# Autodesk Inventor assembly: belt_linear
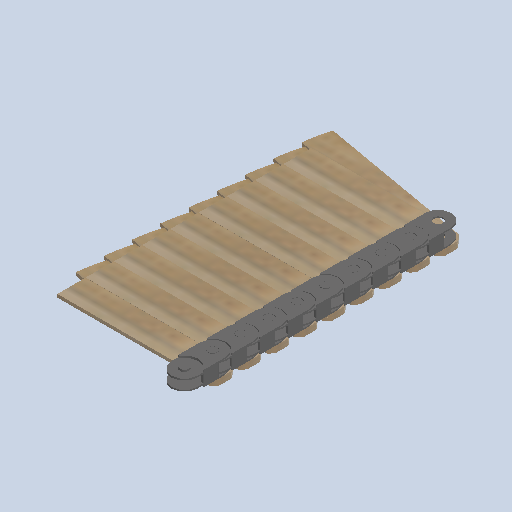
[picture p0: Inventor's stored thumbnail of the model, 512x512]
Saved by Autodesk Inventor 2024.1 (Build 281209000, 209)
## iProperties
Created: 2025-09-27
Part Number: belt_linear
Document SubType Name: Assembly
Designer: hibik
Author: hibik
## Documents named in this file (3)
- C:\Users\hibik\Documents\Robomech\conveyer\belt\belt_linear.iam
- C:\Users\hibik\Documents\Robomech\conveyer\belt\belt.ipt
- C:\Users\hibik\Documents\Robomech\conveyer\belt\dish.iam
## Components (18 placed, 2 different names)
1. belt:1 — 挿入:1, 挿入:5, 角度:1, 角度:9
2. belt:2 — 挿入:1, 挿入:2, 挿入:6, 角度:4, 角度:9, 角度:10
3. belt:3 — 挿入:2, 挿入:3, 挿入:7, 角度:3, 角度:10, 角度:11
4. belt:4 — 挿入:3, 挿入:8, 角度:2, 挿入:16, 角度:11, 角度:12
5. dish:1 [sub-assembly] — 挿入:5, 角度:1
6. dish:2 [sub-assembly] — 挿入:6, 角度:4
7. dish:3 [sub-assembly] — 挿入:7, 角度:3
8. dish:4 [sub-assembly] — 挿入:8, 角度:2
9. belt:5 — 挿入:16, 角度:12, 角度:13
10. belt:6 — 角度:13, 角度:14
11. belt:7 — 角度:14, 角度:15
12. belt:8 — 角度:15, 挿入:18, 角度:17
13. dish:5 [sub-assembly]
14. dish:6 [sub-assembly]
15. dish:7 [sub-assembly]
16. dish:8 [sub-assembly]
17. belt:9 — 挿入:18, 角度:17
18. dish:9 [sub-assembly]
## Relationships (34: Insert 17, Angle 17)
- 挿入:1 [Insert] (0.6 mm): belt:1 ↔ belt:2
- 挿入:2 [Insert] (0.6 mm): belt:2 ↔ belt:3
- 挿入:3 [Insert] (0.6 mm): belt:3 ↔ belt:4
- 挿入:5 [Insert]: belt:1 ↔ dish:1
- 角度:1 [Angle] (0 deg): belt:1 ↔ dish:1
- 挿入:6 [Insert]: belt:2 ↔ dish:2
- 挿入:7 [Insert]: belt:3 ↔ dish:3
- 挿入:8 [Insert]: belt:4 ↔ dish:4
- 角度:2 [Angle] (0 deg): belt:4 ↔ dish:4
- 角度:3 [Angle] (0 deg): belt:3 ↔ dish:3
- 角度:4 [Angle] (0 deg): belt:2 ↔ dish:2
- [Insert] (0.6 mm): belt:5 ↔ belt:6
- [Insert] (0.6 mm): belt:6 ↔ belt:7
- [Insert] (0.6 mm): belt:7 ↔ belt:8
- [Insert]: belt:5 ↔ dish:5
- [Angle] (0 deg): belt:5 ↔ dish:5
- [Insert]: belt:6 ↔ dish:6
- [Insert]: belt:7 ↔ dish:7
- [Insert]: belt:8 ↔ dish:8
- [Angle] (0 deg): belt:8 ↔ dish:8
- [Angle] (0 deg): belt:7 ↔ dish:7
- [Angle] (0 deg): belt:6 ↔ dish:6
- 挿入:16 [Insert] (0.6 mm): belt:4 ↔ belt:5
- 角度:9 [Angle] (0 deg): belt:1 ↔ belt:2
- 角度:10 [Angle] (0 deg): belt:2 ↔ belt:3
- 角度:11 [Angle] (0 deg): belt:3 ↔ belt:4
- 角度:12 [Angle] (0 deg): belt:4 ↔ belt:5
- 角度:13 [Angle] (0 deg): belt:5 ↔ belt:6
- 角度:14 [Angle] (0 deg): belt:6 ↔ belt:7
- 角度:15 [Angle] (0 deg): belt:7 ↔ belt:8
- [Insert]: belt:9 ↔ dish:9
- [Angle] (0 deg): belt:9 ↔ dish:9
- 挿入:18 [Insert] (0.6 mm): belt:8 ↔ belt:9
- 角度:17 [Angle] (0 deg): belt:8 ↔ belt:9
## Named parameters: d12_d0 = 0.6 mm, d13_d1 = 0.6 mm, d14_d2 = 0.6 mm, d15_d4 = 0 mm, d16_d5 = 0 deg, d17_d6 = 0 mm, d18_d7 = 0 mm, d19_d8 = 0 mm, d20_d9 = 0 deg, d21_d10 = 0 deg, d22_d11 = 0 deg, d31_d19_d8 = 0 mm, d32_d20_d9 = 0 deg
